# Autodesk Inventor assembly: case
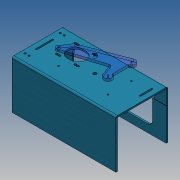
[picture p0: Inventor's stored thumbnail of the model, 180x180]
Saved by Autodesk Inventor 2017 (Build 210142000, 142)
## iProperties
Part Number: case
Material: Genérico
Document SubType Name: Assembly
Designer: Leo
Author: Leo
## Documents named in this file (3)
- C:\Users\Leo\Dropbox\E\Caja Motriz\case.iam
- C:\Users\Leo\Dropbox\E\Caja Motriz\esquema.ipt
- C:\Users\Leo\Dropbox\E\Caja Motriz\Case\Protector.ipt
## Components (2 placed, 2 different names)
1. esquema:1
2. Protector:1 — Nivelación:1, Nivelación:2, Nivelación:3
## Relationships (3: Flush 3)
- Nivelación:1 [Flush] (40 mm): Protector:1
- Nivelación:2 [Flush]: Protector:1
- Nivelación:3 [Flush]: Protector:1
